# Autodesk Inventor assembly: Fuss-1
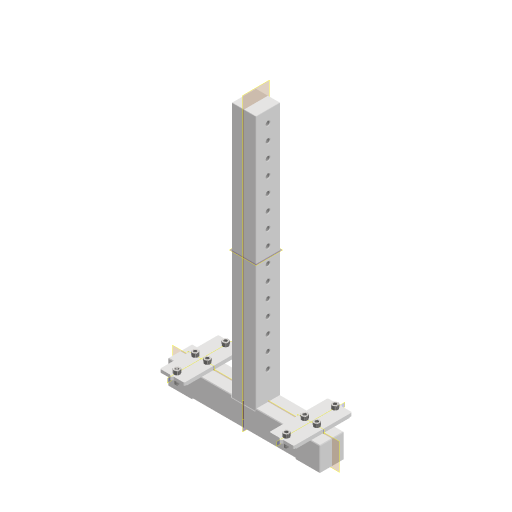
[picture p0: Inventor's stored thumbnail of the model, 512x512]
Saved by Autodesk Inventor 2024.3 (Build 283343000, 343)
## iProperties
Created: 2025-05-16
Part Number: Fuss-1
Document SubType Name: Assembly
Designer: Demir
Author: Demir
## Documents named in this file (7)
- Z:\Verfahreinheit-SWB\Vincent\Fuss.iam
- Z:\Verfahreinheit-SWB\Vincent\Klemmplatte.ipt
- C:\InventorNormteile\Content Center\Libraries\de-DE\DIN 912\DIN 912 - M6 x 1 x 16 x 13,5.ipt
- Z:\Verfahreinheit-SWB\Vincent\Gleitbalken.ipt
- C:\InventorNormteile\Content Center\Libraries\de-DE\DIN 912\DIN 912 - M6 x 1 x 20 x 17,5.ipt
- Z:\Verfahreinheit-SWB\Vincent\Rasterbalken.ipt
- C:\InventorNormteile\Content Center\Libraries\de-DE\DIN 912\DIN 912 - M8 x 1,25 x 40 x 28.ipt
## Components (13 placed, 6 different names)
1. Klemmplatte:1
2. DIN 912 - ersetzt durch DIN EN ISO 4762 M6 x 16:1
3. DIN 912 - ersetzt durch DIN EN ISO 4762 M6 x 16:2
4. DIN 912 - ersetzt durch DIN EN ISO 4762 M6 x 20:1
5. DIN 912 - ersetzt durch DIN EN ISO 4762 M6 x 20:2 — Passend:11
6. Klemmplatte:2
7. DIN 912 - ersetzt durch DIN EN ISO 4762 M6 x 16:3
8. DIN 912 - ersetzt durch DIN EN ISO 4762 M6 x 16:4
9. DIN 912 - ersetzt durch DIN EN ISO 4762 M6 x 20:3
10. DIN 912 - ersetzt durch DIN EN ISO 4762 M6 x 20:4 — Passend:10
11. Gleitbalken:1 — Passend:8, Passend:9, Winkel:1, Passend:10, Passend:11, Einfügen:13
12. Rasterbalken:1 — Passend:8, Passend:9, Winkel:1
13. DIN 912 - ersetzt durch DIN EN ISO 4762 M8 x 40:1 — Einfügen:13
## Relationships (18: Insert 9, Mate 6, Flush 2, Angle 1)
- [Flush]: Klemmplatte:1 ↔ Klemmplatte:2
- [Flush]: Klemmplatte:1 ↔ Klemmplatte:2
- [Insert]: Klemmplatte:1 ↔ DIN 912 - ersetzt durch DIN EN ISO 4762 M6 x 16:1
- [Insert]: Klemmplatte:1 ↔ DIN 912 - ersetzt durch DIN EN ISO 4762 M6 x 16:2
- [Insert]: Klemmplatte:1 ↔ DIN 912 - ersetzt durch DIN EN ISO 4762 M6 x 20:1
- [Insert]: Klemmplatte:1 ↔ DIN 912 - ersetzt durch DIN EN ISO 4762 M6 x 20:2
- [Mate]: Klemmplatte:1 ↔ Gleitbalken:1
- [Mate]: Klemmplatte:1 ↔ Gleitbalken:1
- [Insert]: Klemmplatte:2 ↔ DIN 912 - ersetzt durch DIN EN ISO 4762 M6 x 20:3
- [Insert]: Klemmplatte:2 ↔ DIN 912 - ersetzt durch DIN EN ISO 4762 M6 x 20:4
- [Insert]: Klemmplatte:2 ↔ DIN 912 - ersetzt durch DIN EN ISO 4762 M6 x 16:4
- [Insert]: Klemmplatte:2 ↔ DIN 912 - ersetzt durch DIN EN ISO 4762 M6 x 16:3
- Passend:8 [Mate]: Gleitbalken:1 ↔ Rasterbalken:1
- Passend:9 [Mate]: Gleitbalken:1 ↔ Rasterbalken:1
- Winkel:1 [Angle] (0 deg): Gleitbalken:1 ↔ Rasterbalken:1
- Passend:10 [Mate]: DIN 912 - ersetzt durch DIN EN ISO 4762 M6 x 20:4 ↔ Gleitbalken:1
- Passend:11 [Mate]: DIN 912 - ersetzt durch DIN EN ISO 4762 M6 x 20:2 ↔ Gleitbalken:1
- Einfügen:13 [Insert]: Gleitbalken:1 ↔ DIN 912 - ersetzt durch DIN EN ISO 4762 M8 x 40:1
